# Autodesk Inventor assembly: MTi-1_v3
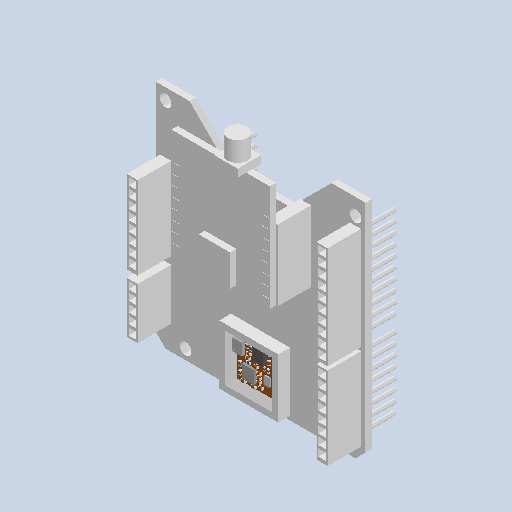
[picture p0: Inventor's stored thumbnail of the model, 512x512]
Saved by Autodesk Inventor 2023 (Build 270158000, 158)
## iProperties
Created: 2023-07-22
Part Number: MTi-1_v3
Description: STEP AP214
Document SubType Name: Assembly
Designer: 310611102
Mass: 8.3834 g
Surface Area: 148.475 cm^2
Volume: 8.3834 cm^3
Density: 1 g/cm^3
Sending System: SolidWorks 2022
Preprocessor: SwSTEP 2.0
Title: MTi-1_v3.STEP
Revision Number: ANY
## Documents named in this file (29)
- C:\Users\310611102\Documents\Inventor\SSR\avionics_2023ver\electronics\MTI-7\MTi 1-series v3.iam
- C:\Users\310611102\Documents\Inventor\SSR\avionics_2023ver\electronics\MTI-7\Board_1v2(2)^MTi-1-SoB_v2.iam
- C:\Users\310611102\Documents\Inventor\SSR\avionics_2023ver\electronics\MTI-7\U200_1v2(2)^MTi-1-SoB_v2.iam
- C:\Users\310611102\Documents\Inventor\SSR\avionics_2023ver\electronics\MTI-7\C200_1v2(2)^MTi-1-SoB_v2.iam
- C:\Users\310611102\Documents\Inventor\SSR\avionics_2023ver\electronics\MTI-7\C201_1v2(2)^MTi-1-SoB_v2.iam
- C:\Users\310611102\Documents\Inventor\SSR\avionics_2023ver\electronics\MTI-7\C204_1v2(2)^MTi-1-SoB_v2.iam
- C:\Users\310611102\Documents\Inventor\SSR\avionics_2023ver\electronics\MTI-7\C205_1v2(2)^MTi-1-SoB_v2.iam
- C:\Users\310611102\Documents\Inventor\SSR\avionics_2023ver\electronics\MTI-7\C206_1v2(2)^MTi-1-SoB_v2.iam
- C:\Users\310611102\Documents\Inventor\SSR\avionics_2023ver\electronics\MTI-7\C207_1v2(2)^MTi-1-SoB_v2.iam
- C:\Users\310611102\Documents\Inventor\SSR\avionics_2023ver\electronics\MTI-7\C208_1v2(2)^MTi-1-SoB_v2.iam
- C:\Users\310611102\Documents\Inventor\SSR\avionics_2023ver\electronics\MTI-7\C209_1v2(2)^MTi-1-SoB_v2.iam
- C:\Users\310611102\Documents\Inventor\SSR\avionics_2023ver\electronics\MTI-7\C300_1v2(2)^MTi-1-SoB_v2.iam
- C:\Users\310611102\Documents\Inventor\SSR\avionics_2023ver\electronics\MTI-7\C301_1v2(2)^MTi-1-SoB_v2.iam
- C:\Users\310611102\Documents\Inventor\SSR\avionics_2023ver\electronics\MTI-7\C302_1v2(2)^MTi-1-SoB_v2.iam
- C:\Users\310611102\Documents\Inventor\SSR\avionics_2023ver\electronics\MTI-7\C303_1v2(2)^MTi-1-SoB_v2.iam
- C:\Users\310611102\Documents\Inventor\SSR\avionics_2023ver\electronics\MTI-7\C305_1v2(2)^MTi-1-SoB_v2.iam
- C:\Users\310611102\Documents\Inventor\SSR\avionics_2023ver\electronics\MTI-7\C304_1v2(2)^MTi-1-SoB_v2.iam
- C:\Users\310611102\Documents\Inventor\SSR\avionics_2023ver\electronics\MTI-7\R200_1v2(2)^MTi-1-SoB_v2.iam
- C:\Users\310611102\Documents\Inventor\SSR\avionics_2023ver\electronics\MTI-7\R300_1v2(2)^MTi-1-SoB_v2.iam
- C:\Users\310611102\Documents\Inventor\SSR\avionics_2023ver\electronics\MTI-7\R301_1v2(2)^MTi-1-SoB_v2.iam
- C:\Users\310611102\Documents\Inventor\SSR\avionics_2023ver\electronics\MTI-7\S300_1v2(2)^MTi-1-SoB_v2.iam
- C:\Users\310611102\Documents\Inventor\SSR\avionics_2023ver\electronics\MTI-7\S301_1v2(2)^MTi-1-SoB_v2.iam
- C:\Users\310611102\Documents\Inventor\SSR\avionics_2023ver\electronics\MTI-7\R302_1v2(2)^MTi-1-SoB_v2.iam
- C:\Users\310611102\Documents\Inventor\SSR\avionics_2023ver\electronics\MTI-7\C202_1v2(2)^MTi-1-SoB_v2.iam
- C:\Users\310611102\Documents\Inventor\SSR\avionics_2023ver\electronics\MTI-7\C203_1v2(2)^MTi-1-SoB_v2.iam
- C:\Users\310611102\Documents\Inventor\SSR\avionics_2023ver\electronics\MTI-7\Y200_1v2(2)^MTi-1-SoB_v2.iam
- C:\Users\310611102\Documents\Inventor\SSR\avionics_2023ver\electronics\MTI-7\R303_1v2(2)^MTi-1-SoB_v2.iam
- C:\Users\310611102\Documents\Inventor\SSR\avionics_2023ver\electronics\MTI-7\Mti-7 development board.ipt
- C:\Users\310611102\Documents\Inventor\SSR\avionics_2023ver\electronics\MTI-7\GNSS_board.ipt
## Components (28 placed, 28 different names)
1. Board_1v2(2)^MTi-1-SoB_v2_1 [sub-assembly] — Mate:1
2. U200_1v2(2)^MTi-1-SoB_v2_2 [sub-assembly]
3. C200_1v2(2)^MTi-1-SoB_v2_3 [sub-assembly]
4. C201_1v2(2)^MTi-1-SoB_v2_4 [sub-assembly]
5. C204_1v2(2)^MTi-1-SoB_v2_5 [sub-assembly]
6. C205_1v2(2)^MTi-1-SoB_v2_6 [sub-assembly]
7. C206_1v2(2)^MTi-1-SoB_v2_7 [sub-assembly]
8. C207_1v2(2)^MTi-1-SoB_v2_8 [sub-assembly]
9. C208_1v2(2)^MTi-1-SoB_v2_9 [sub-assembly]
10. C209_1v2(2)^MTi-1-SoB_v2_10 [sub-assembly]
11. C300_1v2(2)^MTi-1-SoB_v2_11 [sub-assembly]
12. C301_1v2(2)^MTi-1-SoB_v2_12 [sub-assembly]
13. C302_1v2(2)^MTi-1-SoB_v2_13 [sub-assembly]
14. C303_1v2(2)^MTi-1-SoB_v2_14 [sub-assembly]
15. C305_1v2(2)^MTi-1-SoB_v2_15 [sub-assembly]
16. C304_1v2(2)^MTi-1-SoB_v2_16 [sub-assembly]
17. R200_1v2(2)^MTi-1-SoB_v2_17 [sub-assembly]
18. R300_1v2(2)^MTi-1-SoB_v2_18 [sub-assembly]
19. R301_1v2(2)^MTi-1-SoB_v2_19 [sub-assembly]
20. S300_1v2(2)^MTi-1-SoB_v2_20 [sub-assembly]
21. S301_1v2(2)^MTi-1-SoB_v2_21 [sub-assembly]
22. R302_1v2(2)^MTi-1-SoB_v2_22 [sub-assembly]
23. C202_1v2(2)^MTi-1-SoB_v2_23 [sub-assembly]
24. C203_1v2(2)^MTi-1-SoB_v2_24 [sub-assembly]
25. Y200_1v2(2)^MTi-1-SoB_v2_25 [sub-assembly]
26. R303_1v2(2)^MTi-1-SoB_v2_26 [sub-assembly]
27. Mti-7 development board:1 — Mate:1, Mate:2, Mate:3, Mate:4
28. GNSS_board:1 — Mate:2, Mate:3, Mate:4
## Relationships (4: Mate 4)
- Mate:1: Board_1v2(2)^MTi-1-SoB_v2_1 ↔ Mti-7 development board:1
- Mate:2: Mti-7 development board:1 ↔ GNSS_board:1
- Mate:3: Mti-7 development board:1 ↔ GNSS_board:1
- Mate:4: Mti-7 development board:1 ↔ GNSS_board:1
